# Autodesk Inventor assembly: Assembly1
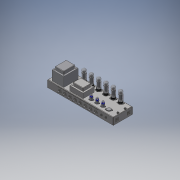
[picture p0: Inventor's stored thumbnail of the model, 180x180]
Saved by Autodesk Inventor 2016 (Build 200138000, 138)
## iProperties
Created: 2015-10-14
Part Number: Assembly1
Document SubType Name: Assembly
Designer: jeremyhale
Author: jeremyhale
## Documents named in this file (31)
- \\psf\Home\Documents\Poorhouse\git\p0001\chassis.iam
- chassis.iam
- \\psf\Home\Documents\Poorhouse\git\p0001\tube socket 8 pin.ipt
- \\psf\Home\Documents\Poorhouse\git\p0001\tube socket 9 pin.ipt
- \\psf\Home\Documents\Poorhouse\git\p0001\xmfr power.ipt
- \\psf\Home\Documents\Poorhouse\git\p0001\xmfr output.ipt
- \\psf\Home\Documents\Inventor\Content Center Files\R2016\en-US\AS 1474(1)\AS 1474 - M3(1).ipt
- \\psf\Home\Documents\Poorhouse\git\p0001\iec320_703W-00_04.ipt
- \\psf\Home\Documents\Inventor\Content Center Files\R2016\en-US\AS 1427(07)\AS 1427 - M3 x 10(6) II.ipt
- \\psf\Home\Documents\Poorhouse\git\p0001\Toggle Large A.ipt
- \\psf\Home\Documents\Poorhouse\git\p0001\AUDIO JACK 2.ipt
- \\psf\Home\Documents\Poorhouse\git\p0001\Bussman fuse holder HKP - 0,25'' X 1,25''.ipt
- \\psf\Home\Documents\Poorhouse\git\p0001\cage nut m6.iam
- \\psf\Home\Documents\Poorhouse\git\p0001\PEC11R-4220F-S0024.ipt
- \\psf\Home\Documents\Inventor\Content Center Files\R2016\en-US\UNI 5590  A\UNI 5590 - A M7.ipt
- \\psf\Home\Documents\Inventor\Content Center Files\R2016\en-US\BS 4320(2)\BS 4320 - M7 (Form B).ipt
- \\psf\Home\Documents\Poorhouse\git\p0001\rotary control.iam
- \\psf\Home\Documents\Poorhouse\git\p0001\Standoff 7mm M2 Wurth 9774070243R.ipt
- \\psf\Home\Documents\Poorhouse\git\p0001\chassis\Design Accelerator\Bolted Connection2.iam
- \\psf\Home\Documents\Poorhouse\git\p0001\chassis\Design Accelerator\Bolted Connection3.iam
- \\psf\Home\Documents\Poorhouse\git\p0001\chassis\Design Accelerator\Bolted Connection4.iam
- \\psf\Home\Documents\Poorhouse\git\p0001\chassis\Design Accelerator\Bolted Connection5.iam
- \\psf\Home\Documents\Poorhouse\git\p0001\chassis\Design Accelerator\Bolted Connection8.iam
- \\psf\Home\Documents\Poorhouse\git\p0001\chassis-weld.iam
- \\psf\Home\Documents\Poorhouse\git\p0001\octal assembly.ipt
- \\psf\Home\Documents\Poorhouse\git\p0001\chassis\Design Accelerator\Bolted Connection6.iam
- \\psf\Home\Documents\Poorhouse\git\p0001\el34 assembly_r1.ipt
- \\psf\Home\Documents\Poorhouse\git\p0001\chassis\Design Accelerator\Bolted Connection7.iam
- \\psf\Home\Documents\Poorhouse\git\p0001\chassis\Design Accelerator\Bolted Connection9.iam
- \\psf\Home\Documents\Poorhouse\git\p0001\Noval socket.ipt
- \\psf\Home\Documents\Poorhouse\git\p0001\12ax7_complete.ipt
## Components (202 placed, 25 different names)
1. xmfr power:1
2. xmfr output:1
3. Bussman fuse holder HKP - 0,25'' X 1,25'':1
4. PowerSwitch
5. chassis-weld:1 [sub-assembly] — Angle:1, Rotational:29, Rotational:30, Insert:43, Angle:2, Rigid:32, Insert:44, Angle:3, Insert:45, Angle:4, Rigid:34
6. big preamp tube socket — Insert:44, Angle:3, Mate:51, Mate:52
7. iec320_703W-00_04:1 — Mate:6, Mate:7
8. AS 1427 Z - Metric M3 x 10:2 — Mate:6, Mate:10
9. AS 1427 Z - Metric M3 x 10:1 — Mate:7, Mate:12
10. AS 1474 - Metric M3:5 — Mate:10
11. AS 1474 - Metric M3:6 — Mate:12
12. cage nut m6:1 [sub-assembly]
13. cage nut m6:2 [sub-assembly]
14. cage nut m6:3 [sub-assembly]
15. cage nut m6:4 [sub-assembly]
16. cage nut m6:5 [sub-assembly]
17. cage nut m6:6 [sub-assembly]
18. cage nut m6:7 [sub-assembly]
19. cage nut m6:8 [sub-assembly]
20. Input Jack
21. AUDIO JACK 2:5
22. Bolted Connection:4 [sub-assembly] — Mate:38
23. Bolted Connection:3 [sub-assembly] — Mate:30
24. Bolted Connection:2 [sub-assembly] — Mate:32
25. Bolted Connection:1 [sub-assembly] — Mate:34
26. Standoff 7mm M2 Wurth 9774070243R:4 — Insert:42, Mate:38
27. Standoff 7mm M2 Wurth 9774070243R:3 — Insert:41, Mate:32
28. Standoff 7mm M2 Wurth 9774070243R:2 — Insert:40, Mate:30
29. Standoff 7mm M2 Wurth 9774070243R:1 — Insert:39, Mate:34
30. rotary control:1 [sub-assembly] — Insert:39, Insert:40, Insert:41, Insert:42, Angle:1, Cylindrical:1, Mate:39, Mate:40
31. BS 4320 Form AB M7 (Form B):1 — Mate:15, Mate:18
32. UNI 5590 A A M7:1 — Mate:17, Mate:18
33. PEC11R-4220F-S0024:1 — Mate:15, Mate:17, Cylindrical:1
34. Bolted Connection:37 [sub-assembly]
35. Bolted Connection:38 [sub-assembly]
36. Bolted Connection:39 [sub-assembly]
37. Bolted Connection:40 [sub-assembly]
38. Standoff 7mm M2 Wurth 9774070243R:5
39. Standoff 7mm M2 Wurth 9774070243R:6
40. Standoff 7mm M2 Wurth 9774070243R:7
41. Standoff 7mm M2 Wurth 9774070243R:8
42. rotary control:2 [sub-assembly]
43. BS 4320 Form AB M7 (Form B):2
44. UNI 5590 A A M7:2
45. PEC11R-4220F-S0024:2
46. Bolted Connection:45 [sub-assembly]
47. Bolted Connection:46 [sub-assembly]
48. Bolted Connection:47 [sub-assembly]
49. Bolted Connection:48 [sub-assembly]
50. Standoff 7mm M2 Wurth 9774070243R:9
51. Standoff 7mm M2 Wurth 9774070243R:10
52. Standoff 7mm M2 Wurth 9774070243R:11
53. Standoff 7mm M2 Wurth 9774070243R:12
54. rotary control:3 [sub-assembly]
55. BS 4320 Form AB M7 (Form B):3
56. UNI 5590 A A M7:3
57. PEC11R-4220F-S0024:3
58. Bolted Connection:53 [sub-assembly]
59. Bolted Connection:54 [sub-assembly]
60. Bolted Connection:55 [sub-assembly]
61. Bolted Connection:56 [sub-assembly]
62. Standoff 7mm M2 Wurth 9774070243R:13
63. Standoff 7mm M2 Wurth 9774070243R:14
64. Standoff 7mm M2 Wurth 9774070243R:15
65. Standoff 7mm M2 Wurth 9774070243R:16
66. rotary control:4 [sub-assembly]
67. BS 4320 Form AB M7 (Form B):4
68. UNI 5590 A A M7:4
69. PEC11R-4220F-S0024:4
70. Bolted Connection:61 [sub-assembly]
71. Bolted Connection:62 [sub-assembly]
72. Bolted Connection:63 [sub-assembly]
73. Bolted Connection:64 [sub-assembly]
74. Standoff 7mm M2 Wurth 9774070243R:17
75. Standoff 7mm M2 Wurth 9774070243R:18
76. Standoff 7mm M2 Wurth 9774070243R:19
77. Standoff 7mm M2 Wurth 9774070243R:20
78. rotary control:5 [sub-assembly]
79. BS 4320 Form AB M7 (Form B):5
80. UNI 5590 A A M7:5
81. PEC11R-4220F-S0024:5
82. Bolted Connection:69 [sub-assembly]
83. Bolted Connection:70 [sub-assembly]
84. Bolted Connection:71 [sub-assembly]
85. Bolted Connection:72 [sub-assembly]
86. Standoff 7mm M2 Wurth 9774070243R:21
87. Standoff 7mm M2 Wurth 9774070243R:22
88. Standoff 7mm M2 Wurth 9774070243R:23
89. Standoff 7mm M2 Wurth 9774070243R:24
90. rotary control:6 [sub-assembly]
91. BS 4320 Form AB M7 (Form B):6
92. UNI 5590 A A M7:6
93. PEC11R-4220F-S0024:6
94. Bolted Connection:77 [sub-assembly]
95. Bolted Connection:78 [sub-assembly]
96. Bolted Connection:79 [sub-assembly]
97. Bolted Connection:80 [sub-assembly]
98. Standoff 7mm M2 Wurth 9774070243R:25
99. Standoff 7mm M2 Wurth 9774070243R:26
100. Standoff 7mm M2 Wurth 9774070243R:27
101. Standoff 7mm M2 Wurth 9774070243R:28
102. rotary control:7 [sub-assembly]
103. BS 4320 Form AB M7 (Form B):7
104. UNI 5590 A A M7:7
105. PEC11R-4220F-S0024:7
106. Bolted Connection:85 [sub-assembly]
107. Bolted Connection:86 [sub-assembly]
108. Bolted Connection:87 [sub-assembly]
109. Bolted Connection:88 [sub-assembly]
110. Standoff 7mm M2 Wurth 9774070243R:29
111. Standoff 7mm M2 Wurth 9774070243R:30
112. Standoff 7mm M2 Wurth 9774070243R:31
113. Standoff 7mm M2 Wurth 9774070243R:32
114. rotary control:8 [sub-assembly]
115. BS 4320 Form AB M7 (Form B):8
116. UNI 5590 A A M7:8
117. PEC11R-4220F-S0024:8
118. AUDIO JACK 2:6 — Rotational:29
119. AUDIO JACK 2:7
120. AUDIO JACK 2:8
121. jack speaker — Rotational:30
122. AUDIO JACK 2:9
123. AUDIO JACK 2:10
124. tube socket 8 pin:1 — Insert:43, Angle:2, Mate:53, Mate:54
125. octal assembly:1 — Rigid:32, Rigid:33
126. el34 assembly_r1:1 — Rigid:33
127. tube socket 8 pin:8
128. octal assembly:2
129. el34 assembly_r1:2
130. tube socket 8 pin:9
131. octal assembly:3
132. el34 assembly_r1:3
133. tube socket 8 pin:10
134. octal assembly:4
135. el34 assembly_r1:4
136. tube socket 8 pin:11
137. octal assembly:5
138. el34 assembly_r1:5
139. tube socket 8 pin:12
140. octal assembly:6
141. el34 assembly_r1:6
142. Bolted Connection:105 [sub-assembly] — Mate:51, Mate:52
143. Bolted Connection:106 [sub-assembly]
144. tube socket 9 pin:1 — Insert:45, Angle:4, Mate:49, Mate:50
145. Noval socket:1 — Rigid:34, Rigid:35
146. 12ax7_complete:1 — Rigid:35
147. tube socket 9 pin:2
148. Noval socket:2
149. 12ax7_complete:2
150. tube socket 9 pin:3
151. Noval socket:3
152. 12ax7_complete:3
153. Bolted Connection:33 [sub-assembly] — Mate:39, Mate:40
154. Bolted Connection:34 [sub-assembly]
155. Bolted Connection:35 [sub-assembly]
156. Bolted Connection:36 [sub-assembly]
157. Bolted Connection:41 [sub-assembly]
158. Bolted Connection:42 [sub-assembly]
159. Bolted Connection:43 [sub-assembly]
160. Bolted Connection:44 [sub-assembly]
161. Bolted Connection:49 [sub-assembly]
162. Bolted Connection:50 [sub-assembly]
163. Bolted Connection:51 [sub-assembly]
164. Bolted Connection:52 [sub-assembly]
165. Bolted Connection:57 [sub-assembly]
166. Bolted Connection:58 [sub-assembly]
167. Bolted Connection:59 [sub-assembly]
168. Bolted Connection:60 [sub-assembly]
169. Bolted Connection:65 [sub-assembly]
170. Bolted Connection:66 [sub-assembly]
171. Bolted Connection:67 [sub-assembly]
172. Bolted Connection:68 [sub-assembly]
173. Bolted Connection:73 [sub-assembly]
174. Bolted Connection:74 [sub-assembly]
175. Bolted Connection:75 [sub-assembly]
176. Bolted Connection:76 [sub-assembly]
177. Bolted Connection:81 [sub-assembly]
178. Bolted Connection:82 [sub-assembly]
179. Bolted Connection:83 [sub-assembly]
180. Bolted Connection:84 [sub-assembly]
181. Bolted Connection:89 [sub-assembly]
182. Bolted Connection:90 [sub-assembly]
183. Bolted Connection:91 [sub-assembly]
184. Bolted Connection:92 [sub-assembly]
185. Bolted Connection:93 [sub-assembly] — Mate:53, Mate:54
186. Bolted Connection:94 [sub-assembly]
187. Bolted Connection:95 [sub-assembly]
188. Bolted Connection:96 [sub-assembly]
189. Bolted Connection:97 [sub-assembly]
190. Bolted Connection:98 [sub-assembly]
191. Bolted Connection:99 [sub-assembly]
192. Bolted Connection:100 [sub-assembly]
193. Bolted Connection:101 [sub-assembly]
194. Bolted Connection:102 [sub-assembly]
195. Bolted Connection:103 [sub-assembly]
196. Bolted Connection:104 [sub-assembly]
197. Bolted Connection:107 [sub-assembly] — Mate:49, Mate:50
198. Bolted Connection:108 [sub-assembly]
199. Bolted Connection:109 [sub-assembly]
200. Bolted Connection:110 [sub-assembly]
201. Bolted Connection:111 [sub-assembly]
202. Bolted Connection:112 [sub-assembly]
## Component patterns: Cage Nuts Top (4 elements), Cage Nuts Right (2 elements), Cage Nuts Left (2 elements), jacks input (2 elements), controls (8 elements), jacks fx (3 elements), jacks speaker (3 elements), big tubes (6 elements), big preamp tube screws (2 elements), small preamp tubes (3 elements), (4 elements, first: Bolted Connection:33), Component Pattern 21:2 (4 elements), Component Pattern 21:3 (4 elements), Component Pattern 21:4 (4 elements), Component Pattern 21:5 (4 elements), Component Pattern 21:6 (4 elements), Component Pattern 21:7 (4 elements), Component Pattern 21:8 (4 elements), big tube socket screws (2 elements), big tube socket screws:2 (2 elements), big tube socket screws:3 (2 elements), big tube socket screws:4 (2 elements), big tube socket screws:5 (2 elements), big tube socket screws:6 (2 elements), small tube screws (2 elements), small tube screws:2 (2 elements), small tube screws:3 (2 elements)
## Relationships (62: Mate 28, RevoluteJoint 10, WeldJoint 9, Insert 7, Angle 4, Flush 3, CylindricalJoint 1)
- [RevoluteJoint]: xmfr power:1 ↔ chassis-weld:1
- [RevoluteJoint]: xmfr power:1 ↔ chassis-weld:1
- [RevoluteJoint]: xmfr output:1 ↔ chassis-weld:1
- [RevoluteJoint]: xmfr output:1 ↔ chassis-weld:1
- [RevoluteJoint]: chassis-weld:1 ↔ iec320_703W-00_04:1
- [RevoluteJoint]: chassis-weld:1 ↔ iec320_703W-00_04:1
- Mate:6: iec320_703W-00_04:1 ↔ AS 1427 Z - Metric M3 x 10:2
- Mate:7: iec320_703W-00_04:1 ↔ AS 1427 Z - Metric M3 x 10:1
- Mate:10: AS 1427 Z - Metric M3 x 10:2 ↔ AS 1474 - Metric M3:5
- [Mate]: chassis-weld:1 ↔ AS 1474 - Metric M3:5
- Mate:12: AS 1427 Z - Metric M3 x 10:1 ↔ AS 1474 - Metric M3:6
- [Mate]: chassis-weld:1 ↔ AS 1474 - Metric M3:6
- [WeldJoint]: Bussman fuse holder HKP - 0,25'' X 1,25'':1 ↔ chassis-weld:1
- [WeldJoint]: PowerSwitch ↔ chassis-weld:1
- [Flush]: chassis-weld:1
- [Flush]: chassis-weld:1
- [Flush]: chassis-weld:1
- [WeldJoint]: chassis-weld:1 ↔ cage nut m6:1
- [WeldJoint]: chassis-weld:1 ↔ cage nut m6:5
- [WeldJoint]: chassis-weld:1 ↔ cage nut m6:7
- Mate:15: BS 4320 Form AB M7 (Form B):1 ↔ PEC11R-4220F-S0024:1
- [Mate]: chassis-weld:1 ↔ BS 4320 Form AB M7 (Form B):1
- Mate:17: UNI 5590 A A M7:1 ↔ PEC11R-4220F-S0024:1
- Mate:18: BS 4320 Form AB M7 (Form B):1 ↔ UNI 5590 A A M7:1
- Insert:39: Standoff 7mm M2 Wurth 9774070243R:1 ↔ rotary control:1
- Insert:40: Standoff 7mm M2 Wurth 9774070243R:2 ↔ rotary control:1
- Insert:41: Standoff 7mm M2 Wurth 9774070243R:3 ↔ rotary control:1
- Insert:42: Standoff 7mm M2 Wurth 9774070243R:4 ↔ rotary control:1
- [Mate]: chassis-weld:1 ↔ Standoff 7mm M2 Wurth 9774070243R:1
- [Mate]: chassis-weld:1 ↔ Standoff 7mm M2 Wurth 9774070243R:4
- Angle:1 (0 deg): chassis-weld:1 ↔ rotary control:1
- Cylindrical:1: rotary control:1 ↔ PEC11R-4220F-S0024:1
- [Mate]: chassis-weld:1 ↔ Bolted Connection:3
- Mate:30: Bolted Connection:3 ↔ Standoff 7mm M2 Wurth 9774070243R:2
- [Mate]: chassis-weld:1 ↔ Bolted Connection:2
- Mate:32: Bolted Connection:2 ↔ Standoff 7mm M2 Wurth 9774070243R:3
- [Mate]: chassis-weld:1 ↔ Bolted Connection:1
- Mate:34: Bolted Connection:1 ↔ Standoff 7mm M2 Wurth 9774070243R:1
- [RevoluteJoint]: chassis-weld:1 ↔ Input Jack
- [RevoluteJoint]: chassis-weld:1 ↔ PEC11R-4220F-S0024:1
- [Mate]: chassis-weld:1 ↔ Bolted Connection:4
- Mate:38: Bolted Connection:4 ↔ Standoff 7mm M2 Wurth 9774070243R:4
- Mate:39: rotary control:1 ↔ Bolted Connection:33
- Mate:40: rotary control:1 ↔ Bolted Connection:33
- Rotational:29 [RevoluteJoint]: chassis-weld:1 ↔ AUDIO JACK 2:6
- Rotational:30 [RevoluteJoint]: chassis-weld:1 ↔ jack speaker
- Insert:43: chassis-weld:1 ↔ tube socket 8 pin:1
- Angle:2 (120 deg): chassis-weld:1 ↔ tube socket 8 pin:1
- Rigid:32 [WeldJoint]: chassis-weld:1 ↔ octal assembly:1
- Rigid:33 [WeldJoint]: octal assembly:1 ↔ el34 assembly_r1:1
- Insert:44: chassis-weld:1 ↔ big preamp tube socket
- Angle:3 (30 deg): chassis-weld:1 ↔ big preamp tube socket
- Insert:45: chassis-weld:1 ↔ tube socket 9 pin:1
- Angle:4 (30 deg): chassis-weld:1 ↔ tube socket 9 pin:1
- Mate:49: tube socket 9 pin:1 ↔ Bolted Connection:107
- Mate:50: tube socket 9 pin:1 ↔ Bolted Connection:107
- Mate:51: big preamp tube socket ↔ Bolted Connection:105
- Mate:52: big preamp tube socket ↔ Bolted Connection:105
- Mate:53: tube socket 8 pin:1 ↔ Bolted Connection:93
- Mate:54: tube socket 8 pin:1 ↔ Bolted Connection:93
- Rigid:34 [WeldJoint]: chassis-weld:1 ↔ Noval socket:1
- Rigid:35 [WeldJoint]: Noval socket:1 ↔ 12ax7_complete:1
## Named parameters: ControlSpacing = 44.45 mm, tubeAngle = 30 deg
